# Autodesk Inventor assembly: Controller Cabinet
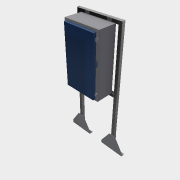
[picture p0: Inventor's stored thumbnail of the model, 180x180]
Saved by Autodesk Inventor 2019.1 (Build 231200000, 200)
## iProperties
Created: 2018-08-31
Part Number: Controller Cabinet
Document SubType Name: Assembly
Designer: alid
Description: Controller Cabinet
Stock Number: NA
Mass: 16079.9 g
Surface Area: 55323.3 cm^2
Volume: 5707.92 cm^3
Density: 2.81712 g/cm^3
_SolveAssemblyDoc: Frame Generator Solve Assembly
_Version: 15.0.0
Author: alid
Title: In House Assembly
Revision Number: A
## Documents named in this file (5)
- C:\Vault Workspace\Process Equipment\Workspace\Options\Controller Cabinet.iam
- C:\Vault Workspace\Process Equipment\Workspace\Framework\SV-Cabinet-Outline.ipt
- C:\Vault Workspace\Process Equipment\Workspace\Framework\SV-Cabinet-Frame\Frame\SV-Cabinet-FR.iam
- C:\Vault Workspace\Process Equipment\Workspace\Supplier Content\P2348-S1-Unistrut.ipt
- C:\Vault Workspace\Process Equipment\Workspace\Components\Control Cabinet Unit.iam
## Components (5 placed, 4 different names)
1. Cabinet_Outline — Flush:1
2. SV-Cabinet-FR:1 [sub-assembly] — Rigid:1, Rigid:2, Flush:2, Mate:1
3. P2348-S1-Unistrut:1 — Rigid:1
4. P2348-S1-Unistrut:2 — Rigid:2
5. Control Cabinet Unit:1 [sub-assembly] — Flush:1, Flush:2, Mate:1
## Relationships (5: WeldJoint 2, Flush 2, Mate 1)
- Rigid:1 [WeldJoint]: SV-Cabinet-FR:1 ↔ P2348-S1-Unistrut:1
- Rigid:2 [WeldJoint]: SV-Cabinet-FR:1 ↔ P2348-S1-Unistrut:2
- Flush:1: Cabinet_Outline ↔ Control Cabinet Unit:1
- Flush:2: SV-Cabinet-FR:1 ↔ Control Cabinet Unit:1
- Mate:1: SV-Cabinet-FR:1 ↔ Control Cabinet Unit:1
